# Autodesk Inventor assembly: GrampoParalelo
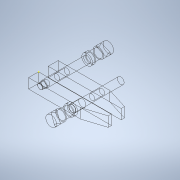
[picture p0: Inventor's stored thumbnail of the model, 180x180]
Saved by Autodesk Inventor 2021 (Build 250183000, 183)
## iProperties
Created: 2022-03-08
Part Number: GrampoParalelo
Document SubType Name: Assembly
Designer: aluno
Author: aluno
## Documents named in this file (5)
- E:\SENAI\Terceiro semestre\TPMC - Tecnololgia de produção mecatrônica\Grampo paralelo\GrampoParalelo.iam
- E:\SENAI\Terceiro semestre\TPMC - Tecnololgia de produção mecatrônica\Grampo paralelo\Garra2.ipt
- E:\SENAI\Terceiro semestre\TPMC - Tecnololgia de produção mecatrônica\Grampo paralelo\Parafuso2.ipt
- E:\SENAI\Terceiro semestre\TPMC - Tecnololgia de produção mecatrônica\Grampo paralelo\Garra1.ipt
- E:\SENAI\Terceiro semestre\TPMC - Tecnololgia de produção mecatrônica\Grampo paralelo\Parafuso1.ipt
## Components (4 placed, 4 different names)
1. Garra2:1 — Coincidente:1, Coincidente:3
2. Parafuso2:1 — Coincidente:1, Inserir:1, Tangente:1
3. Garra1:1 — Inserir:1, Coincidente:2, Coincidente:4, Tangente:1
4. Parafuso1:1 — Coincidente:2, Coincidente:3, Coincidente:4
## Relationships (6: Mate 4, Insert 1, Tangent 1)
- Coincidente:1 [Mate]: Garra2:1 ↔ Parafuso2:1
- Inserir:1: Parafuso2:1 ↔ Garra1:1
- Coincidente:2 [Mate]: Garra1:1 ↔ Parafuso1:1
- Coincidente:3 [Mate]: Garra2:1 ↔ Parafuso1:1
- Coincidente:4 [Mate]: Garra1:1 ↔ Parafuso1:1
- Tangente:1: Parafuso2:1 ↔ Garra1:1
